# Autodesk Inventor assembly: 6P Sprocket
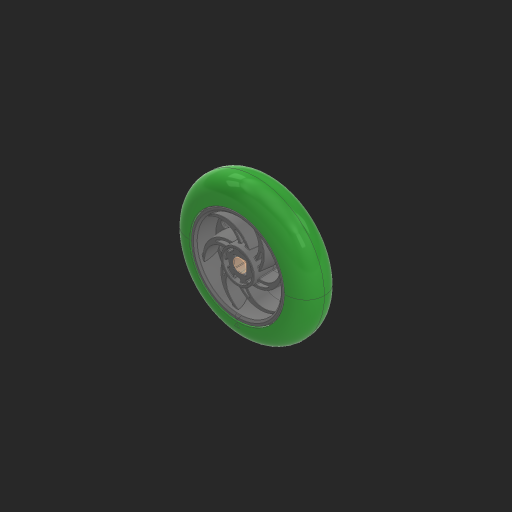
[picture p0: Inventor's stored thumbnail of the model, 512x512]
Saved by Autodesk Inventor 2023 (Build 270158000, 158)
## iProperties
Created: 2022-08-02
Part Number: 6P Sprocket
Document SubType Name: Assembly
Designer: ylu12
Author: ylu12
## Documents named in this file (41)
- C:\Users\ylu12\Documents\GitHub\VEX-CAD-Inventor\Motion\Wheels\Traction Wheel.iam
- C:\Users\ylu12\Documents\GitHub\VEX-CAD-Inventor\Motion\Wheels\Reference Files\2.75 Traction.ipt
- C:\Users\ylu12\Documents\GitHub\VEX-CAD-Inventor\Motion\Wheels\Reference Files\3.25 Traction.ipt
- C:\Users\ylu12\Documents\GitHub\VEX-CAD-Inventor\Motion\Wheels\Reference Files\4 Omni Locked.ipt
- C:\Users\ylu12\Documents\GitHub\VEX-CAD-Inventor\Motion\Wheels\Reference Files\4 Traction.ipt
- C:\Users\ylu12\Documents\GitHub\VEX-CAD-Inventor\Motion\Wheels\Reference Files\4 Traction 169.ipt
- C:\Users\ylu12\Documents\GitHub\VEX-CAD-Inventor\Motion\Wheels\Reference Files\2.75 Traction Antistatic.ipt
- C:\Users\ylu12\Documents\GitHub\VEX-CAD-Inventor\Motion\Wheels\Reference Files\3.25 Traction Antistatic.ipt
- C:\Users\ylu12\Documents\GitHub\VEX-CAD-Inventor\Motion\Wheels\Reference Files\4 Traction Antistatic.ipt
- C:\Users\ylu12\Documents\GitHub\VEX-CAD-Inventor\Motion\Wheels\Reference Files\4 Traction Tire.ipt
- C:\Users\ylu12\Documents\GitHub\VEX-CAD-Inventor\Motion\Insert Circle.ipt
- C:\Users\ylu12\Documents\GitHub\VEX-CAD-Inventor\Motion\Insert Square.ipt
- C:\Users\ylu12\Documents\GitHub\VEX-CAD-Inventor\Motion\HS Shaft Adapter Square.ipt
- C:\Users\ylu12\Documents\GitHub\VEX-CAD-Inventor\Motion\HS Shaft Adapter Circle.ipt
- 169 Traction, Circle.iam
- 169 Traction, No Insert.iam
- 169 Traction, Square.iam
- 2.75 Traction AS, Circle.iam
- 2.75 Traction AS, No Insert.iam
- 2.75 Traction AS, Square.iam
- 2.75 Traction, Circle.iam
- 2.75 Traction, No Insert.iam
- 2.75 Traction, Square.iam
- 3.25 Traction AS, Circle.iam
- 3.25 Traction AS, No Insert.iam
- 3.25 Traction AS, Square.iam
- 3.25 Traction, Circle.iam
- 3.25 Traction, No Insert.iam
- 3.25 Traction, Square.iam
- 4 Omni Locked, Circle.iam
- 4 Omni Locked, No Insert.iam
- 4 Omni Locked, Square.iam
- 4 Traction AS, Circle.iam
- 4 Traction AS, No Insert.iam
- 4 Traction AS, Square.iam
- 4 Traction Tire, Circle.iam
- 4 Traction Tire, No Insert.iam
- 4 Traction Tire, Square.iam
- 4 Traction, Circle.iam
- 4 Traction, No Insert.iam
- 4 Traction, Square.iam
## Components (15 placed, 15 different names)
1. 2.75 Traction — Mate:5, Mate:6, Flush:3
2. 3.25 Traction — Flush:4, Mate:7, Mate:8
3. 4 Omni Locked — Flush:5, Mate:9, Mate:10
4. 4 Traction — Flush:6, Mate:11, Mate:12
5. 169 Traction — Flush:7, Mate:13, Mate:14
6. 2.75 Traction Antistatic:1 — Mate:17, Mate:18, Mate:19
7. 3.25 Traction Antistatic:1 — Mate:20, Mate:22, Mate:24
8. 4 Traction Antistatic:1 — Mate:21, Mate:23, Mate:25
9. 4 Traction Tire:1 — Mate:15, Mate:16, Flush:8
10. Circle 1 — Mate:29, Angle:4, Symmetry:2
11. Square 1 — Mate:28, Angle:2, Symmetry:1
12. Circle 2 — Mate:26, Angle:3, Symmetry:2, Flush:11
13. Square 2 — Mate:27, Angle:1, Symmetry:1, Flush:12
14. Square — Mate:30, Mate:31, Flush:9
15. Circle — Mate:32, Mate:33, Flush:10
## Relationships (45: Mate 29, Flush 10, Angle 4, Symmetry 2)
- Mate:5: 2.75 Traction
- Mate:6: 2.75 Traction
- Flush:3: 2.75 Traction
- Flush:4: 3.25 Traction
- Flush:5: 4 Omni Locked
- Flush:6: 4 Traction
- Flush:7: 169 Traction
- Mate:7: 3.25 Traction
- Mate:8: 3.25 Traction
- Mate:9: 4 Omni Locked
- Mate:10: 4 Omni Locked
- Mate:11: 4 Traction
- Mate:12: 4 Traction
- Mate:13: 169 Traction
- Mate:14: 169 Traction
- Mate:15: 4 Traction Tire:1
- Mate:16: 4 Traction Tire:1
- Flush:8: 4 Traction Tire:1
- Mate:17: 2.75 Traction Antistatic:1
- Mate:18: 2.75 Traction Antistatic:1
- Mate:19: 2.75 Traction Antistatic:1
- Mate:20: 3.25 Traction Antistatic:1
- Mate:21: 4 Traction Antistatic:1
- Mate:22: 3.25 Traction Antistatic:1
- Mate:23: 4 Traction Antistatic:1
- Mate:24: 3.25 Traction Antistatic:1
- Mate:25: 4 Traction Antistatic:1
- Mate:26: Circle 2
- Mate:27: Square 2
- Mate:28: Square 1
- Mate:29: Circle 1
- Angle:1 (0 deg): Square 2
- Angle:2 (0 deg): Square 1
- Angle:3 (0 deg): Circle 2
- Angle:4 (0 deg): Circle 1
- Symmetry:1: Square 1 ↔ Square 2
- Symmetry:2: Circle 1 ↔ Circle 2
- Mate:30: Square
- Mate:31: Square
- Flush:9 (-6.35 mm): Square
- Mate:32: Circle
- Mate:33: Circle
- Flush:10 (6.35 mm): Circle
- Flush:11: Circle 2
- Flush:12 (8.255 mm): Square 2
## Named parameters: Thickness = 8.255 mm
